# Autodesk Inventor assembly: ROBAL_MINI
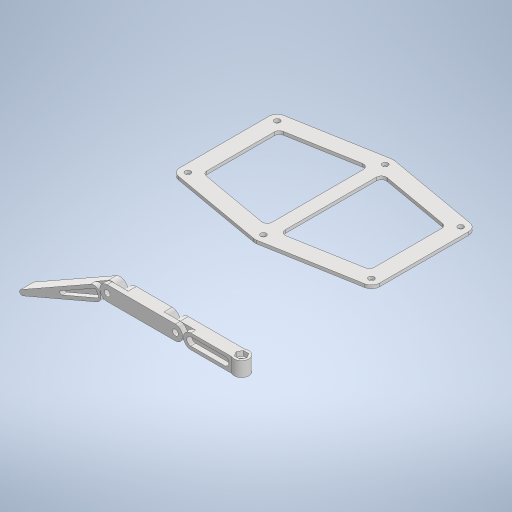
[picture p0: Inventor's stored thumbnail of the model, 512x512]
Saved by Autodesk Inventor 2023 (Build 270158000, 158)
## iProperties
Created: 2024-10-16
Part Number: ROBAL_MINI
Document SubType Name: Assembly
Designer: kamil
Author: kamil
## Documents named in this file (5)
- C:\Users\kamil\Documents\PROJECTS - repos\Robal-2.0\mechanics\mini_robal\ROBAL_MINI.iam
- C:\Users\kamil\Documents\PROJECTS - repos\Robal-2.0\mechanics\mini_robal\L3.ipt
- C:\Users\kamil\Documents\PROJECTS - repos\Robal-2.0\mechanics\mini_robal\L2.ipt
- C:\Users\kamil\Documents\PROJECTS - repos\Robal-2.0\mechanics\mini_robal\L1.ipt
- C:\Users\kamil\Documents\PROJECTS - repos\Robal-2.0\mechanics\mini_robal\podstawa.ipt
## Components (4 placed, 4 different names)
1. L3:1 — Równoległe:1
2. L2:1 — Równoległe:1, Równoległe:2
3. L1:1 — Równoległe:2
4. podstawa:1
## Relationships (2: Flush 2)
- Równoległe:1 [Flush]: L3:1 ↔ L2:1
- Równoległe:2 [Flush]: L2:1 ↔ L1:1
